# Autodesk Inventor assembly: assembledPrototype1-01
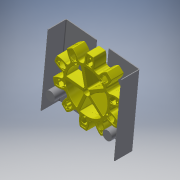
[picture p0: Inventor's stored thumbnail of the model, 180x180]
Saved by Autodesk Inventor 2017 (Build 210142000, 142)
## iProperties
Created: 2017-01-16
Part Number: assembledPrototype1-01
Document SubType Name: Assembly
Designer: kingb
Author: kingb
## Documents named in this file (4)
- C:\Users\kingb\Desktop\CAD\assembledPrototype1-01.iam
- C:\Users\kingb\Desktop\CAD\prototype1(1).ipt
- C:\Users\kingb\Desktop\CAD\scoreGear.iam
- C:\Users\kingb\Desktop\CAD\peg(working).ipt
## Components (4 placed, 3 different names)
1. prototype1(1):1 — Mate:1, Tangent:1, Tangent:2, Mate:2, Mate:3, Tangent:3, Tangent:4
2. scoreGear:1 [sub-assembly] — Mate:1
3. peg(working):1 — Tangent:1, Mate:3, Tangent:4
4. peg(working):2 — Tangent:2, Mate:2, Tangent:3
## Relationships (7: Tangent 4, Mate 3)
- Mate:1: prototype1(1):1 ↔ scoreGear:1
- Tangent:1 (12.7 mm): prototype1(1):1 ↔ peg(working):1
- Tangent:2 (12.7 mm): prototype1(1):1 ↔ peg(working):2
- Mate:2: prototype1(1):1 ↔ peg(working):2
- Mate:3: prototype1(1):1 ↔ peg(working):1
- Tangent:3 (-95.25 mm): prototype1(1):1 ↔ peg(working):2
- Tangent:4 (-95.25 mm): prototype1(1):1 ↔ peg(working):1
